# Autodesk Inventor assembly: intake
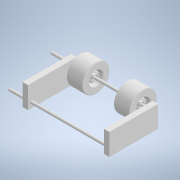
[picture p0: Inventor's stored thumbnail of the model, 180x180]
Saved by Autodesk Inventor 2021 (Build 250183000, 183)
## iProperties
Created: 2020-11-19
Part Number: intake
Document SubType Name: Assembly
Designer: gabe3
Author: gabe3
## Documents named in this file (4)
- D:\robotics\CAD\2020-21-CAD\intake\intake.iam
- D:\robotics\CAD\2020-21-CAD\intake\clolecton wheel holder.ipt
- D:\robotics\CAD\2020-21-CAD\custom parts\.25 axle 9.5in.ipt
- D:\robotics\CAD\COTSParts\Wheels\2.5inFoamWheel250TMD.ipt
## Components (7 placed, 3 different names)
1. clolecton wheel holder:1 — Flush:1, Flush:2, Mate:1, Mate:2, Mate:3
2. clolecton wheel holder:2 — Flush:1, Flush:2, Mate:1, Flush:3
3. .25 axle size template:1 — Mate:2, Flush:3, Flush:4, Mate:4, Mate:5
4. .25 axle size template:2 — Mate:3, Flush:4
5. 2.5inFoamWheel250TMD:1 — Mate:4
6. 2.5inFoamWheel250TMD:2
7. 2.5inFoamWheel250TMD:3 — Mate:5
## Relationships (9: Mate 5, Flush 4)
- Flush:1: clolecton wheel holder:1 ↔ clolecton wheel holder:2
- Flush:2: clolecton wheel holder:1 ↔ clolecton wheel holder:2
- Mate:1 (177.8 mm): clolecton wheel holder:1 ↔ clolecton wheel holder:2
- Mate:2: clolecton wheel holder:1 ↔ .25 axle size template:1
- Flush:3: clolecton wheel holder:2 ↔ .25 axle size template:1
- Mate:3: clolecton wheel holder:1 ↔ .25 axle size template:2
- Flush:4: .25 axle size template:1 ↔ .25 axle size template:2
- Mate:4: .25 axle size template:1 ↔ 2.5inFoamWheel250TMD:1
- Mate:5: .25 axle size template:1 ↔ 2.5inFoamWheel250TMD:3
